# Autodesk Inventor assembly: AssemblyCoxa
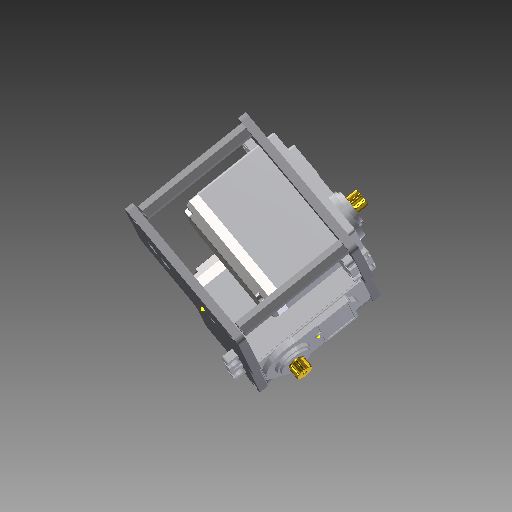
[picture p0: Inventor's stored thumbnail of the model, 512x512]
Saved by Autodesk Inventor 2019 (Build 230136000, 136)
## iProperties
Created: 2023-04-16
Part Number: AssemblyCoxa
Document SubType Name: Assembly
Designer: Analuam
Author: Analuam
## Documents named in this file (9)
- D:\Dek Diyah\AssemblyCoxa.iam
- D:\Dek Diyah\servomg996r\Base.ipt
- D:\Dek Diyah\servomg996r\Eje.ipt
- D:\Dek Diyah\servomg996r\Medio.ipt
- D:\Dek Diyah\servomg996r\Top.ipt
- D:\Dek Diyah\coxa.ipt
- D:\Dek Diyah\coxaa.ipt
- D:\Dek Diyah\Servo berputar.iam
- D:\Dek Diyah\spacer 5cm.ipt
## Components (10 placed, 8 different names)
1. Base:1 — Flush:3, Flush:4, Flush:5, Flush:6, Flush:7, Mate:2
2. Eje:1 — Cylindrical:1, Mate:4
3. Medio:1 — Flush:1, Flush:2, Mate:1, Flush:3, Flush:4, Flush:5, Flush:6, Flush:7, Mate:2, Mate:6
4. Top:1 — Flush:1, Flush:2, Mate:1, Cylindrical:1, Mate:4, Mate:7, Mate:8
5. coxa:1 — Flush:8, Flush:9, Mate:12
6. coxaa:1 — Mate:6, Mate:7, Mate:8, Flush:8, Flush:9, Mate:9, Mate:10, Mate:11, Tangent:1, Mate:13, Mate:14, Mate:15, Insert:1
7. Servo berputar:1 [sub-assembly] — Mate:9, Mate:10, Mate:11, Mate:12
8. spacer 5cm:1 — Tangent:1, Mate:13
9. spacer 5cm:2 — Mate:14, Mate:15
10. spacer 5cm:3 — Insert:1
## Relationships (25: Mate 13, Flush 9, CylindricalJoint 1, Tangent 1, Insert 1)
- Flush:1: Medio:1 ↔ Top:1
- Flush:2: Medio:1 ↔ Top:1
- Mate:1: Medio:1 ↔ Top:1
- Flush:3: Base:1 ↔ Medio:1
- Flush:4: Base:1 ↔ Medio:1
- Flush:5: Base:1 ↔ Medio:1
- Flush:6: Base:1 ↔ Medio:1
- Flush:7: Base:1 ↔ Medio:1
- Mate:2: Base:1 ↔ Medio:1
- Cylindrical:1: Eje:1 ↔ Top:1
- Mate:4: Eje:1 ↔ Top:1
- Mate:6: Medio:1 ↔ coxaa:1
- Mate:7: Top:1 ↔ coxaa:1
- Mate:8: Top:1 ↔ coxaa:1
- Flush:8: coxa:1 ↔ coxaa:1
- Flush:9: coxa:1 ↔ coxaa:1
- Mate:9: coxaa:1 ↔ Servo berputar:1
- Mate:10: coxaa:1 ↔ Servo berputar:1
- Mate:11: coxaa:1 ↔ Servo berputar:1
- Mate:12: coxa:1 ↔ Servo berputar:1
- Tangent:1: coxaa:1 ↔ spacer 5cm:1
- Mate:13: coxaa:1 ↔ spacer 5cm:1
- Mate:14: coxaa:1 ↔ spacer 5cm:2
- Mate:15: coxaa:1 ↔ spacer 5cm:2
- Insert:1: coxaa:1 ↔ spacer 5cm:3
